# Autodesk Inventor assembly: foot pedal
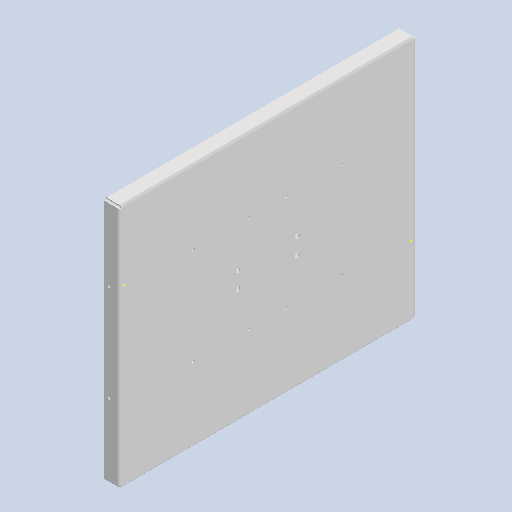
[picture p0: Inventor's stored thumbnail of the model, 512x512]
Saved by Autodesk Inventor 2025.2 (Build 292293000, 293)
## iProperties
Created: 2025-05-20
Part Number: foot pedal
Document SubType Name: Assembly
Designer: Caspe
Mass: 281.11 g
Surface Area: 3804.55 cm^2
Volume: 281.11 cm^3
Density: 1 g/cm^3
Author: Caspe
## Documents named in this file (3)
- C:\Users\Caspe\Documents\Semester 8\Project\Anomaly_Detection\Mechanical_Project\Inventor_project\foot pedal.iam
- C:\Users\Caspe\Documents\Semester 8\Project\Anomaly_Detection\Mechanical_Project\Inventor_project\C_plate V2.ipt
- C:\Users\Caspe\Documents\Semester 8\Project\Anomaly_Detection\Mechanical_Project\Inventor_project\foot_support_V2.ipt
## Components (3 placed, 2 different names)
1. C_plate V2:1 — Insert:1, Insert:2, Insert:3, Insert:4
2. foot_support_V2:1 — Insert:1, Insert:2
3. foot_support_V2:2 — Insert:3, Insert:4
## Relationships (4: Insert 4)
- Insert:1: C_plate V2:1 ↔ foot_support_V2:1
- Insert:2: C_plate V2:1 ↔ foot_support_V2:1
- Insert:3: C_plate V2:1 ↔ foot_support_V2:2
- Insert:4: C_plate V2:1 ↔ foot_support_V2:2
